# Autodesk Inventor assembly: s-assy-scara_link1
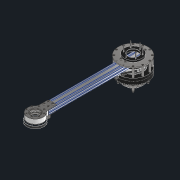
[picture p0: Inventor's stored thumbnail of the model, 180x180]
Saved by Autodesk Inventor 2022 (Build 260153000, 153)
## iProperties
Created: 2021-07-12
Document SubType Name: Assembly
Designer: yuta0
Mass: 2404.35 g
Surface Area: 5708.11 cm^2
Volume: 826.149 cm^3
Density: 2.91031 g/cm^3
Part Number: s-assy-scara_link1
Author: yuta0
## Documents named in this file (14)
- C:\Users\yuta0\Documents\GitHub\catchrobo_hardware\assy-scara\s-assy-scara_link1.iam
- C:\Users\yuta0\Documents\GitHub\catchrobo_hardware\assy-scara\scara-plate1.ipt
- C:\Users\yuta0\Documents\GitHub\catchrobo_hardware\assy-scara\CB5-8.ipt
- C:\Users\yuta0\Documents\GitHub\catchrobo_hardware\assy-scara\scara-base1.ipt
- C:\Users\yuta0\Documents\GitHub\catchrobo_hardware\assy-scara\scara-belt1.ipt
- C:\Users\yuta0\Documents\GitHub\catchrobo_hardware\assy-scara\CB4-40.ipt
- C:\Users\yuta0\Documents\GitHub\catchrobo_hardware\assy-scara\CB4-30.ipt
- C:\Users\yuta0\Documents\GitHub\catchrobo_hardware\assy-scara\CBSTSR4-14.ipt
- C:\Users\yuta0\Documents\GitHub\catchrobo_hardware\assy-scara\HNTT5-5.ipt
- C:\Users\yuta0\Documents\GitHub\catchrobo_hardware\assy-scara\KNFS5-2040_0.ipt
- C:\Users\yuta0\Documents\GitHub\catchrobo_hardware\assy-scara\s-assy-tentioner.iam
- C:\Users\yuta0\Documents\GitHub\catchrobo_hardware\assy-scara\s-assy-outer.iam
- C:\Users\yuta0\Documents\GitHub\catchrobo_hardware\assy-scara\s-assy-scara-unit-j2.iam
- C:\Users\yuta0\Documents\GitHub\catchrobo_hardware\assy-robot\s-assy-unit-j3.iam
## Components (33 placed, 12 different names)
1. KNFS5-2040_0:1 — メイト:172, メイト:188, メイト:215, 角度:1, メイト:263, メイト:266, フラッシュ:4, メイト:267
2. scara-base1:1 — メイト:183, メイト:184, メイト:185, メイト:208, メイト:209, メイト:210, メイト:211
3. scara-plate1:2 — メイト:183, メイト:184, メイト:185, メイト:186, メイト:187, メイト:188, メイト:189, メイト:190, フラッシュ:3, メイト:192, メイト:193, メイト:212, メイト:213, メイト:214
4. s-assy-scara-unit-j2:1 [sub-assembly] — メイト:192, メイト:193, メイト:206, メイト:212, メイト:258
5. scara-belt1:1 — メイト:206, メイト:258, メイト:264, メイト:265, メイト:268
6. CB4-30:1 — メイト:209, メイト:210
7. CB4-30:2 — メイト:208, メイト:211
8. s-assy-tentioner:2 [sub-assembly] — メイト:263, メイト:264, メイト:265
9. s-assy-outer:1 [sub-assembly] — メイト:266, フラッシュ:4, メイト:267, メイト:268
10. CB4-40:1 — メイト:186, メイト:187
11. CB4-40:2
12. CB4-40:3
13. CB4-40:4
14. CB4-40:5
15. CB4-40:6
16. CB5-8:3 — メイト:189, メイト:190, メイト:216
17. HNTT5-5:1 — メイト:215, メイト:216, 角度:1
18. CB5-8:4
19. HNTT5-5:2
20. CB5-8:5
21. HNTT5-5:3
22. CB5-8:6
23. HNTT5-5:4
24. CBSTSR4-14:1 — メイト:213, メイト:214
25. CBSTSR4-14:2
26. CBSTSR4-14:3
27. CBSTSR4-14:4
28. CBSTSR4-14:5
29. CBSTSR4-14:6
30. CBSTSR4-14:7
31. CBSTSR4-14:8
32. CBSTSR4-14:9
33. CBSTSR4-14:10
## Component patterns: (6 elements, first: CB4-40:1), (4 elements, first: CB5-8:3 + HNTT5-5:1), (10 elements, first: CBSTSR4-14:1)
## Relationships (31: Mate 28, Flush 2, Angle 1)
- メイト:172 [Mate]: KNFS5-2040_0:1
- メイト:183 [Mate]: scara-base1:1 ↔ scara-plate1:2
- メイト:184 [Mate]: scara-base1:1 ↔ scara-plate1:2
- メイト:185 [Mate]: scara-base1:1 ↔ scara-plate1:2
- メイト:186 [Mate]: scara-plate1:2 ↔ CB4-40:1
- メイト:187 [Mate]: scara-plate1:2 ↔ CB4-40:1
- メイト:188 [Mate]: KNFS5-2040_0:1 ↔ scara-plate1:2
- メイト:189 [Mate]: scara-plate1:2 ↔ CB5-8:3
- メイト:190 [Mate]: scara-plate1:2 ↔ CB5-8:3
- フラッシュ:3 [Flush]: scara-plate1:2
- メイト:192 [Mate]: scara-plate1:2 ↔ s-assy-scara-unit-j2:1
- メイト:193 [Mate]: scara-plate1:2 ↔ s-assy-scara-unit-j2:1
- メイト:206 [Mate] (0.5 mm): s-assy-scara-unit-j2:1 ↔ scara-belt1:1
- メイト:208 [Mate]: scara-base1:1 ↔ CB4-30:2
- メイト:209 [Mate]: scara-base1:1 ↔ CB4-30:1
- メイト:210 [Mate]: scara-base1:1 ↔ CB4-30:1
- メイト:211 [Mate]: scara-base1:1 ↔ CB4-30:2
- メイト:212 [Mate]: scara-plate1:2 ↔ s-assy-scara-unit-j2:1
- メイト:213 [Mate]: scara-plate1:2 ↔ CBSTSR4-14:1
- メイト:214 [Mate]: scara-plate1:2 ↔ CBSTSR4-14:1
- メイト:215 [Mate]: KNFS5-2040_0:1 ↔ HNTT5-5:1
- メイト:216 [Mate]: CB5-8:3 ↔ HNTT5-5:1
- 角度:1 [Angle] (0 deg): KNFS5-2040_0:1 ↔ HNTT5-5:1
- メイト:258 [Mate]: s-assy-scara-unit-j2:1 ↔ scara-belt1:1
- メイト:263 [Mate]: KNFS5-2040_0:1 ↔ s-assy-tentioner:2
- メイト:264 [Mate]: scara-belt1:1 ↔ s-assy-tentioner:2
- メイト:265 [Mate]: scara-belt1:1 ↔ s-assy-tentioner:2
- メイト:266 [Mate]: KNFS5-2040_0:1 ↔ s-assy-outer:1
- フラッシュ:4 [Flush]: KNFS5-2040_0:1 ↔ s-assy-outer:1
- メイト:267 [Mate]: KNFS5-2040_0:1 ↔ s-assy-outer:1
- メイト:268 [Mate]: scara-belt1:1 ↔ s-assy-outer:1
